# Autodesk Inventor assembly: ARM ASSEMBLY
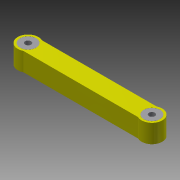
[picture p0: Inventor's stored thumbnail of the model, 180x180]
Saved by Autodesk Inventor 2013 (Build 170138000, 138)
## iProperties
Created: 2013-11-16
Part Number: ARM ASSEMBLY
Document SubType Name: Assembly
Designer: employee
Author: employee
## Documents named in this file (4)
- C:\Users\employee\Desktop\ConceptFORGE\ConceptFORGE\LISA Simpson\INVENTOR FILES\ARM ASSEMBLY.iam
- C:\Users\employee\Desktop\ConceptFORGE\ConceptFORGE\LISA Simpson\INVENTOR FILES\ARM.ipt
- C:\Users\employee\Desktop\ConceptFORGE\ConceptFORGE\LISA Simpson\INVENTOR FILES\_608.ipt
- C:\Users\employee\Desktop\ConceptFORGE\ConceptFORGE\LISA Simpson\INVENTOR FILES\M8 WASHER.ipt
## Components (6 placed, 3 different names)
1. ARM:1 — Insert:1, Insert:2, Insert:3, Insert:4
2. _608:1 — Insert:1
3. _608:2 — Insert:2
4. _608:3 — Insert:3
5. _608:4 — Insert:4, Insert:5
6. M8 WASHER:1 — Insert:5
## Relationships (5: Insert 5)
- Insert:1: ARM:1 ↔ _608:1
- Insert:2: ARM:1 ↔ _608:2
- Insert:3: ARM:1 ↔ _608:3
- Insert:4: ARM:1 ↔ _608:4
- Insert:5: _608:4 ↔ M8 WASHER:1
